# Autodesk Inventor assembly: Übertragung des Zahnriemens
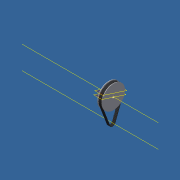
[picture p0: Inventor's stored thumbnail of the model, 180x180]
Saved by Autodesk Inventor 2016 (Build 200138000, 138)
## iProperties
Created: 2016-02-16
Part Number: Übertragung des Zahnriemens
Document SubType Name: Assembly
Designer: 4ndreas
Mass: 21.673 g
Surface Area: 100.997 cm^2
Volume: 20.5857 cm^3
Density: 1.05282 g/cm^3
ClientObjectVersion: 1
Author: 4ndreas
## Documents named in this file (3)
- C:\Users\4ndreas\Documents\github\Mantis-Robot-Arm\MantisRobotArm\Workspace\_Wrist_rev1\Wrist_r1\Konstruktions-Assistent\Übertragung des Zahnriemens1.iam
- C:\Users\4ndreas\Documents\github\Mantis-Robot-Arm\MantisRobotArm\Workspace\_Wrist_rev1\Wrist_r1\Konstruktions-Assistent\Zahnriemen1.ipt
- C:\Users\4ndreas\Documents\github\Mantis-Robot-Arm\MantisRobotArm\Workspace\_Wrist_rev1\Wrist_r1\Konstruktions-Assistent\Synchrone Riemenscheibe21.ipt
## Components (2 placed, 2 different names)
1. Zahnriemen:1 — Fluchtend:1, Passend:1, Passend:2
2. Synchrone Riemenscheibe2:1 — Fluchtend:1, Passend:1, Passend:2
## Relationships (3: Mate 2, Flush 1)
- Fluchtend:1 [Flush]: Zahnriemen:1 ↔ Synchrone Riemenscheibe2:1
- Passend:1 [Mate]: Zahnriemen:1 ↔ Synchrone Riemenscheibe2:1
- Passend:2 [Mate]: Zahnriemen:1 ↔ Synchrone Riemenscheibe2:1
